# Autodesk Inventor assembly: ChainLinks
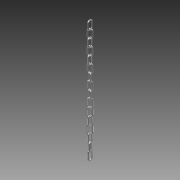
[picture p0: Inventor's stored thumbnail of the model, 180x180]
Saved by Autodesk Inventor 2013 (Build 170138000, 138)
## iProperties
Shininess: 0.0
Length Units: 11272
Angle Units: 11279
Time Units: 11290
Mass Units: 11286
Length Display Precision: 3
Angle Display Precision: 2
Compacted: True
Created: 2000-09-30
Part Number: ChainLinks
Document SubType Name: Assembly
Designer: Administrator
Density: 0.0
Volumn: 0.0
Area: 0.0
PropertySet Name: Model Information
Control State: 0
Master: False
Checked Out: False
Author: Administrator
## Documents named in this file (2)
- E:\Data Folder\FIRST 2013\FIRST KOP\FIRST Arena 2013\Pyramid\chain.iam
- E:\Data Folder\FIRST 2013\FIRST KOP\FIRST Arena 2013\Pyramid\3-16 link.ipt
## Components (16 placed, 1 different names)
1. 3-16 link:1 — Mate:1, Angle:1, Mate:10, Angle:10, Angle:27, Angle:28
2. 3-16 link:2 — Mate:1, Mate:2, Angle:1, Angle:2, Angle:26, Angle:27
3. 3-16 link:3 — Mate:2, Mate:3, Angle:2, Angle:5, Angle:23, Angle:25, Angle:26
4. 3-16 link:4 — Mate:3, Mate:4, Angle:3, Angle:5, Angle:23, Angle:24, Angle:25
5. 3-16 link:5 — Mate:4, Mate:5, Angle:3, Angle:4, Angle:22, Angle:24
6. 3-16 link:6 — Mate:5, Angle:4, Angle:6, Mate:9, Angle:21, Angle:22
7. 3-16 link:7 — Mate:8, Angle:6, Angle:7, Mate:9, Angle:20, Angle:21
8. 3-16 link:8 — Mate:6, Mate:8, Angle:7, Angle:8, Angle:19, Angle:20
9. 3-16 link:9 — Mate:6, Mate:7, Angle:8, Angle:9, Angle:18, Angle:19
10. 3-16 link:10 — Mate:7, Angle:9, Angle:18
11. 3-16 link:11 — Mate:10, Mate:11, Angle:10, Angle:11, Angle:28, Angle:29
12. 3-16 link:12 — Mate:11, Mate:12, Angle:11, Angle:12, Angle:29, Angle:30
13. 3-16 link:13 — Mate:12, Angle:12, Mate:13, Angle:13, Angle:30, Angle:31
14. 3-16 link:14 — Mate:13, Angle:13, Mate:14, Angle:14, Angle:31, Angle:32
15. 3-16 link:15 — Mate:14, Angle:14, Mate:15, Angle:15, Angle:32, Angle:33
16. 3-16 link:16 — Mate:15, Angle:15, Angle:33
## Relationships (46: Angle 31, Mate 15)
- Mate:1: 3-16 link:1 ↔ 3-16 link:2
- Mate:2: 3-16 link:2 ↔ 3-16 link:3
- Mate:3: 3-16 link:3 ↔ 3-16 link:4
- Mate:4: 3-16 link:4 ↔ 3-16 link:5
- Mate:5: 3-16 link:5 ↔ 3-16 link:6
- Angle:1 (30 deg): 3-16 link:1 ↔ 3-16 link:2
- Angle:2 (30 deg): 3-16 link:2 ↔ 3-16 link:3
- Angle:3 (30 deg): 3-16 link:4 ↔ 3-16 link:5
- Angle:4 (30 deg): 3-16 link:5 ↔ 3-16 link:6
- Mate:6: 3-16 link:8 ↔ 3-16 link:9
- Mate:7: 3-16 link:9 ↔ 3-16 link:10
- Mate:8: 3-16 link:7 ↔ 3-16 link:8
- Angle:5 (30 deg): 3-16 link:3 ↔ 3-16 link:4
- Angle:6 (30 deg): 3-16 link:6 ↔ 3-16 link:7
- Angle:7 (30 deg): 3-16 link:7 ↔ 3-16 link:8
- Angle:8 (30 deg): 3-16 link:8 ↔ 3-16 link:9
- Angle:9 (30 deg): 3-16 link:9 ↔ 3-16 link:10
- Mate:9: 3-16 link:6 ↔ 3-16 link:7
- Mate:10: 3-16 link:1 ↔ 3-16 link:11
- Mate:11: 3-16 link:11 ↔ 3-16 link:12
- Mate:12: 3-16 link:12 ↔ 3-16 link:13
- Angle:10 (30 deg): 3-16 link:1 ↔ 3-16 link:11
- Angle:11 (30 deg): 3-16 link:11 ↔ 3-16 link:12
- Angle:12 (30 deg): 3-16 link:12 ↔ 3-16 link:13
- Mate:13: 3-16 link:13 ↔ 3-16 link:14
- Angle:13 (30 deg): 3-16 link:13 ↔ 3-16 link:14
- Mate:14: 3-16 link:14 ↔ 3-16 link:15
- Angle:14 (30 deg): 3-16 link:14 ↔ 3-16 link:15
- Mate:15: 3-16 link:15 ↔ 3-16 link:16
- Angle:15 (30 deg): 3-16 link:15 ↔ 3-16 link:16
- Angle:18 (0 deg): 3-16 link:9 ↔ 3-16 link:10
- Angle:19 (0 deg): 3-16 link:8 ↔ 3-16 link:9
- Angle:20 (0 deg): 3-16 link:7 ↔ 3-16 link:8
- Angle:21 (0 deg): 3-16 link:6 ↔ 3-16 link:7
- Angle:22 (0 deg): 3-16 link:5 ↔ 3-16 link:6
- Angle:23 (0 deg): 3-16 link:3 ↔ 3-16 link:4
- Angle:24 (0 deg): 3-16 link:4 ↔ 3-16 link:5
- Angle:25 (0 deg): 3-16 link:3 ↔ 3-16 link:4
- Angle:26 (0 deg): 3-16 link:2 ↔ 3-16 link:3
- Angle:27 (0 deg): 3-16 link:1 ↔ 3-16 link:2
- Angle:28 (0 deg): 3-16 link:1 ↔ 3-16 link:11
- Angle:29 (0 deg): 3-16 link:11 ↔ 3-16 link:12
- Angle:30 (0 deg): 3-16 link:12 ↔ 3-16 link:13
- Angle:31 (0 deg): 3-16 link:13 ↔ 3-16 link:14
- Angle:32 (0 deg): 3-16 link:14 ↔ 3-16 link:15
- Angle:33 (0 deg): 3-16 link:15 ↔ 3-16 link:16
## Named parameters: chain_angle = 30 deg
